# Autodesk Inventor assembly: syncNew
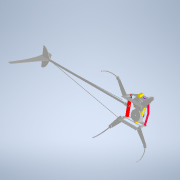
[picture p0: Inventor's stored thumbnail of the model, 180x180]
Saved by Autodesk Inventor 2020 (Build 240168000, 168)
## iProperties
Created: 2019-06-16
Part Number: syncNew
Document SubType Name: Assembly
Designer: Vivek Muskan
Author: Vivek Muskan
## Documents named in this file (23)
- C:\Users\Vivek Muskan\Documents\TARGET25\syncNew.iam
- C:\Users\Vivek Muskan\Documents\TARGET25\DLFinal.ipt
- C:\Users\Vivek Muskan\Documents\TARGET25\centralFinal.ipt
- C:\Users\Vivek Muskan\Documents\TARGET25\SIdeFinal.ipt
- C:\Users\Vivek Muskan\Documents\TARGET25\servo.ipt
- C:\Users\Vivek Muskan\Documents\TARGET25\kundi.ipt
- C:\Users\Vivek Muskan\Documents\TARGET25\mount.ipt
- C:\Users\Vivek Muskan\Documents\TARGET25\spacerFinal.iam
- C:\Users\Vivek Muskan\Documents\TARGET25\angularPlate.ipt
- C:\Users\Vivek Muskan\Documents\TARGET25\MotorSupport.ipt
- C:\Users\Vivek Muskan\Documents\TARGET25\connector.ipt
- C:\Users\Vivek Muskan\Documents\TARGET25\plateHolder.ipt
- C:\Users\Vivek Muskan\Documents\TARGET25\plateHolder2.ipt
- C:\Users\Vivek Muskan\Documents\TARGET25\plateLocker.ipt
- C:\Users\Vivek Muskan\Documents\TARGET25\prependicular.ipt
- C:\Users\Vivek Muskan\Documents\TARGET25\connectotr_Mirror.ipt
- C:\Users\Vivek Muskan\Documents\TARGET25\plateLockerMirror.ipt
- C:\Users\Vivek Muskan\Documents\TARGET25\arm.ipt
- C:\Users\Vivek Muskan\Documents\TARGET25\armMirror.ipt
- C:\Users\Vivek Muskan\Documents\TARGET25\tail.ipt
- C:\Users\Vivek Muskan\Documents\TARGET25\rodHolder.ipt
- C:\Users\Vivek Muskan\Documents\TARGET25\shortSpaver.ipt
- C:\Users\Vivek Muskan\Documents\TARGET25\preBuiltArm.ipt
## Components (58 placed, 22 different names)
1. DLFinal:1 — Flush:3, Mate:2, Flush:4, Mate:3, Angle:1
2. centralFinal:1 — Mate:1, Flush:1, Flush:2, Symmetry:1, Flush:4, Mate:7, Mate:9, Mate:10, Mate:11, Flush:5, Flush:6, Mate:28, Mate:29, Mate:30, Mate:31, Flush:9, Mate:32, Mate:40, Mate:42, Mate:63, Insert:33, Insert:34
3. centralFinal:2 — Mate:1, Flush:1, Flush:2, Symmetry:1, Mate:2, Mate:5, Mate:6, Mate:8, Mate:18, Mate:33, Mate:37, Mate:43, Mate:44, Mate:45, Mate:49, Mate:50, Mate:70, Mate:71, Mate:72, Flush:11, Mate:73, Mate:74
4. SIdeFinal:1 — Mate:5, Mate:7, Mate:20, Insert:3, Insert:4, Flush:6, Mate:26, Mate:27, Mate:34, Mate:38, Mate:39, Mate:52, Mate:53, Mate:55, Mate:56, Mate:57, Mate:58, Mate:59, Insert:9, Insert:10, Insert:31, Insert:32, Insert:43, Insert:44
5. SIdeFinal:2 — Mate:6, Mate:8, Mate:19, Insert:1, Insert:2, Flush:5, Mate:35, Mate:36, Mate:46, Mate:47, Mate:48, Mate:51, Mate:54, Mate:60, Mate:61, Mate:62, Insert:7, Insert:8, Insert:45, Insert:46
6. servo:1 — Mate:37, Mate:38, Mate:39
7. servo:3 — Mate:9, Mate:10, Mate:11
8. servo:6 — Mate:18, Mate:49, Mate:50
9. kundi:1 — Mate:19, Insert:1, Insert:2
10. kundi:2 — Mate:20, Insert:3, Insert:4
11. mount:1 — Mate:23, Flush:7, Flush:8, Mate:27, Mate:28
12. mount:2 — Mate:23, Flush:7, Flush:8, Mate:26
13. spacerFinal:1 [sub-assembly] — Flush:9, Mate:32, Mate:33
14. spacerFinal:4 [sub-assembly] — Mate:29, Mate:30, Mate:31
15. servo:7 — Mate:40, Mate:42, Mate:63
16. servo:8 — Mate:46, Mate:47, Mate:48
17. servo:9 — Mate:43, Mate:44, Mate:45
18. angularPlate:1 — Mate:54, Mate:55, Mate:56, Insert:73, Insert:74, Insert:75
19. angularPlate:2 — Mate:51, Mate:52, Mate:53, Insert:72
20. MotorSupport:1 — Mate:57, Mate:58, Mate:59
21. MotorSupport:2 — Mate:60, Mate:61, Mate:62
22. connector:1 — Insert:7, Insert:8, Insert:37, Insert:38, Insert:48, Flush:12, Mate:75, Flush:13
23. connector:3 — Insert:9, Insert:10, Insert:53, Insert:54, Insert:62, Flush:14, Flush:15, Mate:76
24. spacerFinal:5 [sub-assembly] — Flush:11, Mate:73, Mate:74
25. spacerFinal:6 [sub-assembly] — Mate:70, Mate:71, Mate:72
26. kundi:3 — Insert:31, Insert:32
27. kundi:4 — Insert:33, Insert:34
28. plateLocker:2 — Insert:37, Insert:38, Insert:40, Insert:42, Insert:47
29. plateHolder:2 — Insert:40, Insert:50
30. plateHolder2:1 — Insert:42
31. prependicular:1 — Insert:68, Flush:16, Mate:78
32. prependicular:2 — Insert:55, Flush:15
33. prependicular:3 — Insert:69, Insert:70
34. prependicular:4 — Insert:48, Insert:65, Flush:12
35. prependicular:5 — Insert:47, Flush:13
36. connectotr_Mirror:1 — Insert:45, Insert:46, Insert:49, Flush:16, Insert:69, Mate:77
37. connectotr_Mirror:2 — Insert:43, Insert:44, Insert:56, Insert:57, Insert:64, Mate:79, Flush:17, Flush:18
38. plateLockerMirror:1 — Insert:53, Insert:54, Insert:55, Insert:58, Insert:60
39. plateLockerMirror:2 — Insert:49, Insert:50, Insert:68
40. plateLocker:3 — Insert:56, Insert:57, Insert:59, Insert:61, Insert:63
41. plateHolder:3 — Insert:58, Insert:59
42. plateHolder2:2 — Insert:60, Insert:61
43. prependicular:6 — Insert:62, Flush:14, Insert:66
44. prependicular:7 — Insert:63, Flush:17
45. prependicular:9 — Insert:64, Insert:71, Flush:18
46. arm:1 — Insert:65, Mate:75, Insert:78
47. arm:2 — Insert:66, Mate:76, Insert:80
48. armMirror:1 — Insert:71, Mate:79, Insert:81
49. armMirror:2 — Insert:70, Mate:77, Mate:78, Insert:79
50. tail:1 — Insert:72
51. rodHolder:1 — Insert:76, Insert:77
52. shortSpaver:1 — Insert:73
53. shortSpaver:2 — Insert:74, Insert:77
54. shortSpaver:3 — Insert:75, Insert:76
55. preBuiltArm:1 — Insert:78
56. preBuiltArm:2 — Insert:81
57. preBuiltArm:3 — Insert:80
58. preBuiltArm:4 — Insert:79
## Relationships (133: Mate 62, Insert 52, Flush 17, Symmetry 1, Angle 1)
- Mate:1 (50 mm): centralFinal:1 ↔ centralFinal:2
- Flush:1: centralFinal:1 ↔ centralFinal:2
- Flush:2: centralFinal:1 ↔ centralFinal:2
- Symmetry:1: centralFinal:1 ↔ centralFinal:2
- Flush:3: DLFinal:1
- Mate:2 (26.5 mm): DLFinal:1 ↔ centralFinal:2
- Flush:4: DLFinal:1 ↔ centralFinal:1
- Mate:3: DLFinal:1
- Mate:4
- Angle:1 (90 deg): DLFinal:1
- Mate:5: centralFinal:2 ↔ SIdeFinal:1
- Mate:6: centralFinal:2 ↔ SIdeFinal:2
- Mate:7: centralFinal:1 ↔ SIdeFinal:1
- Mate:8: centralFinal:2 ↔ SIdeFinal:2
- Mate:9: centralFinal:1 ↔ servo:3
- Mate:10: centralFinal:1 ↔ servo:3
- Mate:11: centralFinal:1 ↔ servo:3
- Mate:18: centralFinal:2 ↔ servo:6
- Mate:19: SIdeFinal:2 ↔ kundi:1
- Insert:1: SIdeFinal:2 ↔ kundi:1
- Insert:2: SIdeFinal:2 ↔ kundi:1
- Mate:20: SIdeFinal:1 ↔ kundi:2
- Insert:3: SIdeFinal:1 ↔ kundi:2
- Insert:4: SIdeFinal:1 ↔ kundi:2
- Flush:5: centralFinal:1 ↔ SIdeFinal:2
- Flush:6: centralFinal:1 ↔ SIdeFinal:1
- Mate:23: mount:1 ↔ mount:2
- Flush:7: mount:1 ↔ mount:2
- Flush:8: mount:1 ↔ mount:2
- Mate:26: SIdeFinal:1 ↔ mount:2
- Mate:27: SIdeFinal:1 ↔ mount:1
- Mate:28: centralFinal:1 ↔ mount:1
- Mate:29: centralFinal:1 ↔ spacerFinal:4
- Mate:30: centralFinal:1 ↔ spacerFinal:4
- Mate:31: centralFinal:1 ↔ spacerFinal:4
- Flush:9: centralFinal:1 ↔ spacerFinal:1
- Mate:32: centralFinal:1 ↔ spacerFinal:1
- Mate:33: centralFinal:2 ↔ spacerFinal:1
- Mate:34: SIdeFinal:1
- Mate:35: SIdeFinal:2
- Mate:36: SIdeFinal:2
- Mate:37: centralFinal:2 ↔ servo:1
- Mate:38: SIdeFinal:1 ↔ servo:1
- Mate:39: SIdeFinal:1 ↔ servo:1
- Mate:40: centralFinal:1 ↔ servo:7
- Mate:42: centralFinal:1 ↔ servo:7
- Mate:43: centralFinal:2 ↔ servo:9
- Mate:44: centralFinal:2 ↔ servo:9
- Mate:45: centralFinal:2 ↔ servo:9
- Mate:46: SIdeFinal:2 ↔ servo:8
- Mate:47: SIdeFinal:2 ↔ servo:8
- Mate:48: SIdeFinal:2 ↔ servo:8
- Mate:49: centralFinal:2 ↔ servo:6
- Mate:50: centralFinal:2 ↔ servo:6
- Mate:51: SIdeFinal:2 ↔ angularPlate:2
- Mate:52: SIdeFinal:1 ↔ angularPlate:2
- Mate:53: SIdeFinal:1 ↔ angularPlate:2
- Mate:54: SIdeFinal:2 ↔ angularPlate:1
- Mate:55: SIdeFinal:1 ↔ angularPlate:1
- Mate:56: SIdeFinal:1 ↔ angularPlate:1
- Mate:57: SIdeFinal:1 ↔ MotorSupport:1
- Mate:58: SIdeFinal:1 ↔ MotorSupport:1
- Mate:59: SIdeFinal:1 ↔ MotorSupport:1
- Mate:60: SIdeFinal:2 ↔ MotorSupport:2
- Mate:61: SIdeFinal:2 ↔ MotorSupport:2
- Mate:62: SIdeFinal:2 ↔ MotorSupport:2
- Insert:7: SIdeFinal:2 ↔ connector:1
- Insert:8: SIdeFinal:2 ↔ connector:1
- Insert:9: SIdeFinal:1 ↔ connector:3
- Insert:10: SIdeFinal:1 ↔ connector:3
- Mate:63: centralFinal:1 ↔ servo:7
- Mate:70: centralFinal:2 ↔ spacerFinal:6
- Mate:71: centralFinal:2 ↔ spacerFinal:6
- Mate:72: centralFinal:2 ↔ spacerFinal:6
- Flush:11: centralFinal:2 ↔ spacerFinal:5
- Mate:73: centralFinal:2 ↔ spacerFinal:5
- Mate:74: centralFinal:2 ↔ spacerFinal:5
- Insert:31: SIdeFinal:1 ↔ kundi:3
- Insert:32: SIdeFinal:1 ↔ kundi:3
- Insert:33: centralFinal:1 ↔ kundi:4
- Insert:34: centralFinal:1 ↔ kundi:4
- Insert:37: connector:1 ↔ plateLocker:2
- Insert:38: connector:1 ↔ plateLocker:2
- Insert:40: plateLocker:2 ↔ plateHolder:2
- Insert:42: plateLocker:2 ↔ plateHolder2:1
- Insert:43: SIdeFinal:1 ↔ connectotr_Mirror:2
- Insert:44: SIdeFinal:1 ↔ connectotr_Mirror:2
- Insert:45: SIdeFinal:2 ↔ connectotr_Mirror:1
- Insert:46: SIdeFinal:2 ↔ connectotr_Mirror:1
- Insert:47: plateLocker:2 ↔ prependicular:5
- Insert:48: connector:1 ↔ prependicular:4
- Insert:49: connectotr_Mirror:1 ↔ plateLockerMirror:2
- Insert:50: plateHolder:2 ↔ plateLockerMirror:2
- Insert:53: connector:3 ↔ plateLockerMirror:1
- Insert:54: connector:3 ↔ plateLockerMirror:1
- Insert:55: prependicular:2 ↔ plateLockerMirror:1
- Insert:56: connectotr_Mirror:2 ↔ plateLocker:3
- Insert:57: connectotr_Mirror:2 ↔ plateLocker:3
- Insert:58: plateLockerMirror:1 ↔ plateHolder:3
- Insert:59: plateLocker:3 ↔ plateHolder:3
- Insert:60: plateLockerMirror:1 ↔ plateHolder2:2
- Insert:61: plateLocker:3 ↔ plateHolder2:2
- Insert:62: connector:3 ↔ prependicular:6
- Insert:63: plateLocker:3 ↔ prependicular:7
- Insert:64: connectotr_Mirror:2 ↔ prependicular:9
- Insert:65: prependicular:4 ↔ arm:1
- Flush:12 (1.5 mm): connector:1 ↔ prependicular:4
- Mate:75: connector:1 ↔ arm:1
- Flush:13: connector:1 ↔ prependicular:5
- Flush:14 (1.5 mm): connector:3 ↔ prependicular:6
- Flush:15: connector:3 ↔ prependicular:2
- Insert:66: prependicular:6 ↔ arm:2
- Mate:76: connector:3 ↔ arm:2
- Insert:68: prependicular:1 ↔ plateLockerMirror:2
- Flush:16: prependicular:1 ↔ connectotr_Mirror:1
- Insert:69: prependicular:3 ↔ connectotr_Mirror:1
- Insert:70: prependicular:3 ↔ armMirror:2
- Mate:77: connectotr_Mirror:1 ↔ armMirror:2
- Mate:78: prependicular:1 ↔ armMirror:2
- Insert:71: prependicular:9 ↔ armMirror:1
- Mate:79: connectotr_Mirror:2 ↔ armMirror:1
- Flush:17: connectotr_Mirror:2 ↔ prependicular:7
- Flush:18 (1.5 mm): connectotr_Mirror:2 ↔ prependicular:9
- Insert:72: angularPlate:2 ↔ tail:1
- Insert:73: angularPlate:1 ↔ shortSpaver:1
- Insert:74: angularPlate:1 ↔ shortSpaver:2
- Insert:75: angularPlate:1 ↔ shortSpaver:3
- Insert:76: rodHolder:1 ↔ shortSpaver:3
- Insert:77: rodHolder:1 ↔ shortSpaver:2
- Insert:78: arm:1 ↔ preBuiltArm:1
- Insert:79: armMirror:2 ↔ preBuiltArm:4
- Insert:80: arm:2 ↔ preBuiltArm:3
- Insert:81: armMirror:1 ↔ preBuiltArm:2
